# Autodesk Inventor assembly: boltnuttopassembly
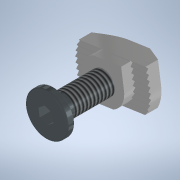
[picture p0: Inventor's stored thumbnail of the model, 180x180]
Saved by Autodesk Inventor 2020.2 (Build 242310000, 310)
## iProperties
Created: 2020-07-25
Part Number: boltnuttopassembly
Document SubType Name: Assembly
Designer: JK
Author: JK
## Documents named in this file (3)
- C:\Users\JK\Documents\Inventor\Mesa\boltnuttopassembly.iam
- C:\Users\JK\Documents\Inventor\Mesa\M5x15BoltFlatHead.ipt
- C:\Users\JK\Documents\Inventor\Mesa\T_Slot_Nut_Dropin_3030m5ipt.ipt
## Components (2 placed, 2 different names)
1. M5x15BoltFlatHead:1 — Mate:1, Angle:1, Mate:2
2. T_Slot_Nut_Dropin_3030m5ipt:1 — Mate:1, Angle:1, Mate:2
## Relationships (3: Mate 2, Angle 1)
- Mate:1: M5x15BoltFlatHead:1 ↔ T_Slot_Nut_Dropin_3030m5ipt:1
- Angle:1 (0 deg): M5x15BoltFlatHead:1 ↔ T_Slot_Nut_Dropin_3030m5ipt:1
- Mate:2 (12.5 mm): M5x15BoltFlatHead:1 ↔ T_Slot_Nut_Dropin_3030m5ipt:1
